# Autodesk Inventor assembly: cart_assembly
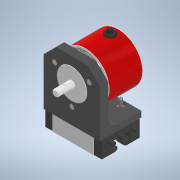
[picture p0: Inventor's stored thumbnail of the model, 180x180]
Saved by Autodesk Inventor 2021 (Build 250183000, 183)
## iProperties
Created: 2022-07-01
Part Number: cart_assembly
Document SubType Name: Assembly
Designer: lenna
Author: lenna
## Documents named in this file (9)
- C:\Users\lenna\Desktop\Lennart\Uni\Master\2. Semester\SDM\CAD_neu\cart_assembly.iam
- C:\Users\lenna\Desktop\Lennart\Uni\Master\2. Semester\SDM\CAD_neu\cart.ipt
- C:\Users\lenna\Desktop\Lennart\Uni\Master\2. Semester\SDM\CAD_neu\encoder_adapter.ipt
- C:\Users\lenna\Desktop\Lennart\Uni\Master\2. Semester\SDM\CAD_neu\opkon_encoder.ipt
- C:\Users\lenna\Desktop\Lennart\Uni\Master\2. Semester\SDM\CAD_neu\M3_tread_insert.ipt
- C:\Users\lenna\Documents\Inventor\Content Center Files\R2021\en-US\DIN EN ISO 4035\DIN EN ISO 4035 - M4.ipt
- C:\Users\lenna\Documents\Inventor\Content Center Files\R2021\en-US\ISO 4762(1)\DIN EN ISO 4762 - M4 x 30.ipt
- C:\Users\lenna\Documents\Inventor\Content Center Files\R2021\en-US\ISO 4762(1)\DIN EN ISO 4762 - M3 x 25.ipt
- C:\Users\lenna\Documents\Inventor\Content Center Files\R2021\en-US\ISO 4762(1)\DIN EN ISO 4762 - M3 x 10.ipt
## Components (14 placed, 8 different names)
1. cart:1 — Flush:1, Flush:2, Flush:3, Insert:1, Insert:2, Insert:9, Insert:10
2. encoder_adapter:1 — Insert:1, Insert:2, Insert:3, Mate:1, Insert:5, Insert:6, Insert:8
3. opkon_encoder:1 — Insert:3, Mate:1
4. DIN EN ISO 4762 M3 x 10:1 — Insert:8
5. DIN EN ISO 4762 M3 x 10:2
6. DIN EN ISO 4762 M3 x 10:3
7. DIN EN ISO 4762 M3 x 25:1 — Insert:9
8. M3_tread_insert:2 — Insert:5
9. DIN EN ISO 4762 M4 x 30:1 — Insert:10
10. DIN EN ISO 4035 M4:1 — Insert:6
11. DIN EN ISO 4762 M3 x 25:2
12. M3_tread_insert:3
13. DIN EN ISO 4762 M4 x 30:2
14. DIN EN ISO 4035 M4:2
## Component patterns: (3 elements, first: DIN EN ISO 4762 M3 x 10:1), (2 elements, first: DIN EN ISO 4762 M3 x 25:1 + M3_tread_insert:2 + DIN EN ISO 4762 M4 x 30:1 + DIN EN ISO 4035 M4:1)
## Relationships (12: Insert 8, Flush 3, Mate 1)
- Flush:1: cart:1
- Flush:2: cart:1
- Flush:3: cart:1
- Insert:1: cart:1 ↔ encoder_adapter:1
- Insert:2: cart:1 ↔ encoder_adapter:1
- Insert:3: encoder_adapter:1 ↔ opkon_encoder:1
- Mate:1: encoder_adapter:1 ↔ opkon_encoder:1
- Insert:5: encoder_adapter:1 ↔ M3_tread_insert:2
- Insert:6: encoder_adapter:1 ↔ DIN EN ISO 4035 M4:1
- Insert:8: encoder_adapter:1 ↔ DIN EN ISO 4762 M3 x 10:1
- Insert:9: cart:1 ↔ DIN EN ISO 4762 M3 x 25:1
- Insert:10: cart:1 ↔ DIN EN ISO 4762 M4 x 30:1
